# Autodesk Inventor assembly: Ensamble cilindro
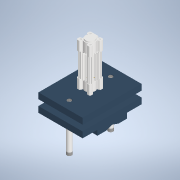
[picture p0: Inventor's stored thumbnail of the model, 180x180]
Saved by Autodesk Inventor 2021 (Build 250183000, 183)
## iProperties
Created: 2021-04-29
Part Number: Ensamble cilindro
Document SubType Name: Assembly
Designer: Admin
Author: Admin
## Documents named in this file (7)
- C:\Users\Nelson\Github\Proyecto_APM\Inventor_Corte\Ensamble cilindro.iam
- C:\Users\Nelson\Github\Proyecto_APM\Inventor_Corte\Soporte Superior Tubos.ipt
- C:\Users\Nelson\Github\Proyecto_APM\Inventor_Corte\Soporte Pistón.ipt
- C:\Users\Nelson\Github\Proyecto_APM\Inventor_Corte\AIS2021\CP96SDB32-50-M9P(0_0_0).iam
- D:\Nelson\Documentos\Inventor\Content Center Files\R2021\en-US\DIN 7984\DIN 7984 - M8 x 25.ipt
- C:\Users\Nelson\Github\Proyecto_APM\Inventor_Corte\DIN 7984 - M8 x 25.ipt
- C:\Users\Nelson\Github\Proyecto_APM\Inventor_Corte\Eje roscado base soporte tubo.ipt
## Components (7 placed, 5 different names)
1. CP96SDB32-50-M9P(0_0_0):1 [sub-assembly] — Mate:122, Mate:123, Mate:138, Mate:141, Mate:142, Mate:143
2. Soporte Superior Tubos:1 — Mate:122, Mate:123
3. Soporte Pistón:1 — Mate:138, Mate:141, Mate:142, Mate:143, Mate:146, Mate:147, Mate:148, Mate:149, Mate:151, Mate:152, Mate:155
4. DIN 7984 M8 x 25:1 — Mate:147, Mate:149
5. DIN 7984 M8 x 25:2 — Mate:146, Mate:148, Mate:150
6. Eje roscado base soporte tubo:1 — Mate:150, Mate:152
7. Eje roscado base soporte tubo:2 — Mate:151, Mate:155
## Relationships (15: Mate 15)
- [Mate]: CP96SDB32-50-M9P(0_0_0):1 ↔ Soporte Superior Tubos:1
- Mate:122: CP96SDB32-50-M9P(0_0_0):1 ↔ Soporte Superior Tubos:1
- Mate:123: CP96SDB32-50-M9P(0_0_0):1 ↔ Soporte Superior Tubos:1
- Mate:138: CP96SDB32-50-M9P(0_0_0):1 ↔ Soporte Pistón:1
- Mate:141: CP96SDB32-50-M9P(0_0_0):1 ↔ Soporte Pistón:1
- Mate:142: CP96SDB32-50-M9P(0_0_0):1 ↔ Soporte Pistón:1
- Mate:143: CP96SDB32-50-M9P(0_0_0):1 ↔ Soporte Pistón:1
- Mate:146: Soporte Pistón:1 ↔ DIN 7984 M8 x 25:2
- Mate:147: Soporte Pistón:1 ↔ DIN 7984 M8 x 25:1
- Mate:148: Soporte Pistón:1 ↔ DIN 7984 M8 x 25:2
- Mate:149: Soporte Pistón:1 ↔ DIN 7984 M8 x 25:1
- Mate:150: DIN 7984 M8 x 25:2 ↔ Eje roscado base soporte tubo:1
- Mate:151: Soporte Pistón:1 ↔ Eje roscado base soporte tubo:2
- Mate:152: Soporte Pistón:1 ↔ Eje roscado base soporte tubo:1
- Mate:155: Soporte Pistón:1 ↔ Eje roscado base soporte tubo:2
